# Autodesk Inventor assembly: Frame
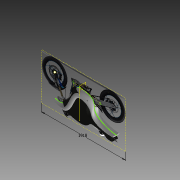
[picture p0: Inventor's stored thumbnail of the model, 180x180]
Saved by Autodesk Inventor 2016 (Build 200138000, 138)
## iProperties
Created: 2015-03-25
Part Number: Frame
Document SubType Name: Assembly
Designer: Yann
Author: Yann
## Documents named in this file (7)
- C:\Users\Yann\Documents\GitHub\BIKAIR_CAD\Source\Frame\Frame.iam
- C:\Users\Yann\Documents\GitHub\BIKAIR_CAD\Source\Frame\Frame_Generator.ipt
- C:\Users\Yann\Documents\GitHub\BIKAIR_CAD\Source\Frame\Seat.iam
- C:\Users\Yann\Documents\GitHub\BIKAIR_CAD\Source\Frame\Shell.ipt
- C:\Users\Yann\Documents\GitHub\BIKAIR_CAD\Source\Frame\Master.ipt
- C:\Users\Yann\Documents\GitHub\BIKAIR_CAD\Source\Frame\Pivots_Support.ipt
- C:\Program Files (x86)\Common Files\Autodesk Shared\Materials\Textures\carbon-fiber--very-detailed.jpg
## Components (5 placed, 5 different names)
1. Shell:1 — Flush:3, Flush:4, Flush:5
2. Frame_Generator:1 — Affleurement:2, Placage:1, Placage:2
3. Seat:1 [sub-assembly]
4. Master:1
5. Pivots_Support:1
## Relationships (6: Flush 4, Mate 2)
- Affleurement:2 [Flush]: Frame_Generator:1
- Placage:1 [Mate]: Frame_Generator:1
- Placage:2 [Mate]: Frame_Generator:1
- Flush:3: Shell:1
- Flush:4: Shell:1
- Flush:5: Shell:1
